# Autodesk Inventor assembly: obudowa - budzik v3.3
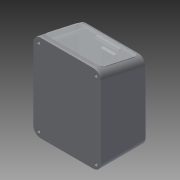
[picture p0: Inventor's stored thumbnail of the model, 180x180]
Saved by Autodesk Inventor 2014 (Build 180170000, 170)
## iProperties
Created: 2018-03-05
Part Number: obudowa - budzik v3.3
Document SubType Name: Assembly
Designer: HP820
Author: HP820
## Documents named in this file (4)
- C:\Users\HP820\Dysk Google\Projekt SYSTEM POWIADOMIEN DLA OSOB GLUCHONIEMYCH I NIEDOSLYSZACYCH BY JACEK MARTYNIAK I ŁUKASZ NOWARKIEWICZ\Projekty 3D obudowy\obudowa - budzik\obudowa - budzik v3.3.iam
- C:\Users\HP820\Dysk Google\Projekt SYSTEM POWIADOMIEN DLA OSOB GLUCHONIEMYCH I NIEDOSLYSZACYCH BY JACEK MARTYNIAK I ŁUKASZ NOWARKIEWICZ\Projekty 3D obudowy\obudowa - budzik\obudowa - budzik v3 dol.ipt
- C:\Users\HP820\Dysk Google\Projekt SYSTEM POWIADOMIEN DLA OSOB GLUCHONIEMYCH I NIEDOSLYSZACYCH BY JACEK MARTYNIAK I ŁUKASZ NOWARKIEWICZ\Projekty 3D obudowy\obudowa - budzik\obudowa - budzik v3 plexi.ipt
- C:\Users\HP820\Dysk Google\Projekt SYSTEM POWIADOMIEN DLA OSOB GLUCHONIEMYCH I NIEDOSLYSZACYCH BY JACEK MARTYNIAK I ŁUKASZ NOWARKIEWICZ\Projekty 3D obudowy\obudowa - budzik\obudowa - budzik v3 dol dol.ipt
## Components (3 placed, 3 different names)
1. obudowa - budzik v3 dol:1 — Flush:1, Flush:2
2. obudowa - budzik v3 plexi:1 — Flush:1
3. obudowa - budzik v3 dol dol:1 — Flush:2
## Relationships (2: Flush 2)
- Flush:1: obudowa - budzik v3 dol:1 ↔ obudowa - budzik v3 plexi:1
- Flush:2: obudowa - budzik v3 dol:1 ↔ obudowa - budzik v3 dol dol:1
